# Autodesk Inventor assembly: sheetA
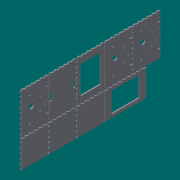
[picture p0: Inventor's stored thumbnail of the model, 180x180]
Saved by Autodesk Inventor 2016 SP2 (Build 200236200, 236)
## iProperties
Created: 2016-09-27
Part Number: sheetA
Document SubType Name: Assembly
Designer: sawaiz
Author: sawaiz
## Documents named in this file (8)
- C:\Users\sawaiz\OneDrive\projects\splitFlapDisplay\sheetA.iam
- C:\Users\sawaiz\oneDrive\projects\splitFlapDisplay\frame\leftSide.ipt
- C:\Users\sawaiz\oneDrive\projects\splitFlapDisplay\frame\back.ipt
- C:\Users\sawaiz\oneDrive\projects\splitFlapDisplay\frame\front.ipt
- C:\Users\sawaiz\oneDrive\projects\splitFlapDisplay\frame\topBottomPanel.ipt
- C:\Users\sawaiz\oneDrive\projects\splitFlapDisplay\frame\rightSide.ipt
- C:\Users\sawaiz\oneDrive\projects\splitFlapDisplay\sheetA.ipt
- C:\Users\sawaiz\oneDrive\projects\splitFlapDisplay\parameters.xlsx
## Components (10 placed, 6 different names)
1. leftSide:1 — Flush:1, Flush:2, Flush:3, Flush:4, Flush:5, Flush:10, Mate:3, Flush:13, Mate:5, Flush:19
2. back:1 — Flush:3, Flush:5, Flush:6, Flush:9, Flush:10, Mate:2, Mate:3
3. front:1 — Flush:2, Flush:6, Flush:7, Mate:1, Flush:8, Flush:9, Mate:2, Flush:15
4. topBottomPanel:1 — Flush:4, Flush:13, Mate:5, Flush:14, Flush:16, Mate:6
5. rightSide:1 — Flush:1, Flush:7, Mate:1, Flush:8, Flush:11, Flush:12, Mate:4, Flush:18, Mate:8, Flush:20
6. leftSide:2 — Flush:11, Flush:12, Mate:4
7. topBottomPanel:2 — Flush:14, Flush:16, Flush:17, Mate:6, Mate:7
8. topBottomPanel:3 — Flush:15, Flush:17, Mate:7, Mate:9
9. front:2 — Flush:18, Mate:8, Mate:9
10. sheetA:1 — Flush:19, Flush:20
## Relationships (29: Flush 20, Mate 9)
- Flush:1: leftSide:1 ↔ rightSide:1
- Flush:2: leftSide:1 ↔ front:1
- Flush:3: leftSide:1 ↔ back:1
- Flush:4: leftSide:1 ↔ topBottomPanel:1
- Flush:5: leftSide:1 ↔ back:1
- Flush:6: back:1 ↔ front:1
- Flush:7: front:1 ↔ rightSide:1
- Mate:1 (0.36 mm): front:1 ↔ rightSide:1
- Flush:8: front:1 ↔ rightSide:1
- Flush:9: back:1 ↔ front:1
- Flush:10: leftSide:1 ↔ back:1
- Mate:2 (0.36 mm): back:1 ↔ front:1
- Mate:3 (0.36 mm): leftSide:1 ↔ back:1
- Flush:11: rightSide:1 ↔ leftSide:2
- Flush:12: rightSide:1 ↔ leftSide:2
- Mate:4 (0.36 mm): rightSide:1 ↔ leftSide:2
- Flush:13: leftSide:1 ↔ topBottomPanel:1
- Mate:5 (0.36 mm): leftSide:1 ↔ topBottomPanel:1
- Flush:14: topBottomPanel:1 ↔ topBottomPanel:2
- Flush:15: front:1 ↔ topBottomPanel:3
- Flush:16: topBottomPanel:1 ↔ topBottomPanel:2
- Flush:17: topBottomPanel:2 ↔ topBottomPanel:3
- Mate:6 (0.36 mm): topBottomPanel:1 ↔ topBottomPanel:2
- Mate:7 (0.36 mm): topBottomPanel:2 ↔ topBottomPanel:3
- Flush:18: rightSide:1 ↔ front:2
- Mate:8 (0.36 mm): rightSide:1 ↔ front:2
- Mate:9 (0.36 mm): topBottomPanel:3 ↔ front:2
- Flush:19: leftSide:1 ↔ sheetA:1
- Flush:20: rightSide:1 ↔ sheetA:1
## Named parameters: height = 180 mm, width = 120 mm, depth = 120 mm, materialThickness = 3.175 mm, laserKerf = 0.12 mm, spoolDiameter = 90 mm, cardPinDiameter = 3 mm, cardNumber = 40, centeralShaftDiameter = 8 mm, cardWidth = 85.6 mm, cardHeight = 53.98 mm, cardThickness = 0.76 mm, cardFillet = 2.88 mm, cardCutoutHeight = 20 mm, cardClearence = 0.5 mm, spoolHubDiameter = 20 mm, bearingOd = 22 mm, bearingWidth = 8 mm, axleHeight = 95 mm, nutTrapClearence = 2 mm, nutTrapwidth = 5.5 mm, nutTrapDepth = 2.5 mm, beltLength = 240 mm, magnetDiameter = 6 mm, magnetLength = 3 mm, magnetProtusion = 0.25 mm, notchWidth = 10 mm, spoolThickness = 5.588 mm
